# Autodesk Inventor assembly: Small Limit Switch
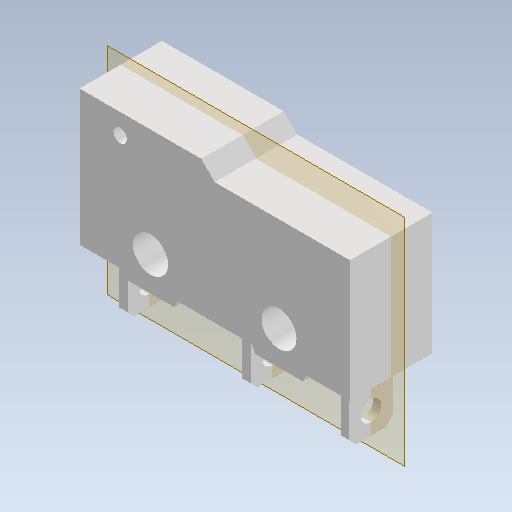
[picture p0: Inventor's stored thumbnail of the model, 512x512]
Saved by Autodesk Inventor 2022 (Build 260153000, 153)
## iProperties
Created: 2019-04-17
Part Number: Small Limit Switch
Document SubType Name: Assembly
Designer: Parker
Mass: 1.13155 g
Surface Area: 9.50399 cm^2
Volume: 1.13155 cm^3
Density: 1 g/cm^3
Author: Parker
## Documents named in this file (2)
- D:\Designs\MK3PRO P1\COMPONENTS\Small Limit Switch.iam
- D:\Designs\MK3PRO P1\COMPONENTS\Small Limit Switch\Body.ipt
## Components (1 placed, 1 different names)
1. Body:1 — Flush:3
## Relationships (1: Flush 1)
- Flush:3 (-3.05 mm): Body:1
